# Autodesk Inventor assembly: Ensamblaje carcasa control
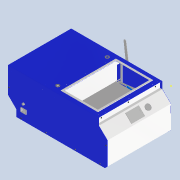
[picture p0: Inventor's stored thumbnail of the model, 180x180]
Saved by Autodesk Inventor 2021 (Build 250183000, 183)
## iProperties
Created: 2021-04-15
Part Number: Ensamblaje carcasa control
Document SubType Name: Assembly
Designer: Admin
Author: Admin
## Documents named in this file (21)
- E:\Documentos\Documentos\Michael_Rodriguez\Universidad_Nacional\Doceaba matricula\PAI\Proyecto PAI\Proyecto_PAI_2021\01 CAD\Ensamblaje carcasa control.iam
- E:\Documentos\Documentos\Michael_Rodriguez\Universidad_Nacional\Doceaba matricula\PAI\Proyecto PAI\Proyecto_PAI_2021\01 CAD\Carcasa_azul.ipt
- E:\Documentos\Documentos\Michael_Rodriguez\Universidad_Nacional\Doceaba matricula\PAI\Proyecto PAI\Proyecto_PAI_2021\01 CAD\Carcaza_blanca_frontal.ipt
- E:\Documentos\Documentos\Michael_Rodriguez\Universidad_Nacional\Doceaba matricula\PAI\Proyecto PAI\Proyecto_PAI_2021\01 CAD\Tapa_blanca_inferior.ipt
- E:\Documentos\Documentos\Michael_Rodriguez\Universidad_Nacional\Doceaba matricula\PAI\Proyecto PAI\Proyecto_PAI_2021\01 CAD\Vacuometro.ipt
- E:\Documentos\Documentos\Michael_Rodriguez\Universidad_Nacional\Doceaba matricula\PAI\Proyecto PAI\Proyecto_PAI_2021\01 CAD\HMI_NV3W_MR20L_V1.iam
- E:\Documentos\Documentos\Michael_Rodriguez\Universidad_Nacional\Doceaba matricula\PAI\Proyecto PAI\Proyecto_PAI_2021\01 CAD\Receptaculo e interruptor.ipt
- E:\Documentos\Documentos\Michael_Rodriguez\Universidad_Nacional\Doceaba matricula\PAI\Proyecto PAI\Proyecto_PAI_2021\01 CAD\Portafusible para fusible de 13A.ipt
- E:\Documentos\Documentos\Michael_Rodriguez\Universidad_Nacional\Doceaba matricula\PAI\Proyecto PAI\Proyecto_PAI_2021\01 CAD\Tapa_interior_1.ipt
- E:\Documentos\Documentos\Michael_Rodriguez\Universidad_Nacional\Doceaba matricula\PAI\Proyecto PAI\Proyecto_PAI_2021\01 CAD\Tapa_interior_2.ipt
- E:\Documentos\Documentos\Michael_Rodriguez\Universidad_Nacional\Doceaba matricula\PAI\Proyecto PAI\Proyecto_PAI_2021\01 CAD\Tapa_blanca_trasera.ipt
- E:\Documentos\Documentos\Michael_Rodriguez\Universidad_Nacional\Doceaba matricula\PAI\Proyecto PAI\Proyecto_PAI_2021\01 CAD\Ensamble eléctrico.iam
- E:\Documentos\Documentos\Michael_Rodriguez\Universidad_Nacional\Doceaba matricula\PAI\Proyecto PAI\Proyecto_PAI_2021\01 CAD\Bomba de Vacio.ipt
- E:\Documentos\Documentos\Michael_Rodriguez\Universidad_Nacional\Doceaba matricula\PAI\Proyecto PAI\Proyecto_PAI_2021\01 CAD\Marco molde.ipt
- E:\Documentos\Documentos\Michael_Rodriguez\Universidad_Nacional\Doceaba matricula\PAI\Proyecto PAI\Proyecto_PAI_2021\01 CAD\CSN 02 1721 - 17,5.ipt
- E:\Documentos\Documentos\Michael_Rodriguez\Universidad_Nacional\Doceaba matricula\PAI\Proyecto PAI\Proyecto_PAI_2021\01 CAD\Ensamblaje_soportme molde_barras.iam
- E:\Documentos\Documentos\Michael_Rodriguez\Universidad_Nacional\Doceaba matricula\PAI\Proyecto PAI\Proyecto_PAI_2021\01 CAD\Mecanismo Modelado.iam
- E:\Documentos\Documentos\Michael_Rodriguez\Universidad_Nacional\Doceaba matricula\PAI\Proyecto PAI\Proyecto_PAI_2021\01 CAD\Bandeja_proteccion_carcasa_control.ipt
- E:\Documentos\Documentos\Michael_Rodriguez\Universidad_Nacional\Doceaba matricula\PAI\Proyecto PAI\Proyecto_PAI_2021\01 CAD\BS 4320 - M5 (Forma A).ipt
- E:\Documentos\Documentos\Michael_Rodriguez\Universidad_Nacional\Doceaba matricula\PAI\Proyecto PAI\Proyecto_PAI_2021\01 CAD\ISO 7380-1 - M5 x 8.ipt
- E:\Documentos\Documentos\Michael_Rodriguez\Universidad_Nacional\Doceaba matricula\PAI\Proyecto PAI\Proyecto_PAI_2021\01 CAD\BS 4183 - M5(1).ipt
## Components (81 placed, 20 different names)
1. Carcasa_azul:1 — Coincidencia:1, Nivelación:1, Coincidencia:2, Coincidencia:3, Nivelación:2, Coincidencia:5, Coincidencia:6, Coincidencia:7, Coincidencia:8, Coincidencia:9, Coincidencia:15, Coincidencia:16, Coincidencia:18, Coincidencia:20, Coincidencia:27, Nivelación:6, Nivelación:7, Coincidencia:28, Coincidencia:29, Coincidencia:30, Coincidencia:31, Coincidencia:32, Coincidencia:33, Coincidencia:34, Nivelación:8, Nivelación:9, Coincidencia:35, De rotación:1, De rotación:2, De rotación:3, De rotación:4, De rotación:5, De rotación:6, De rotación:7, De rotación:8, De rotación:9, De rotación:10, De rotación:11, De rotación:12, De rotación:42, De rotación:43, De rotación:47, De rotación:48
2. Carcaza_blanca_frontal:1 — Coincidencia:1, Nivelación:1, Coincidencia:2, Coincidencia:4, Coincidencia:10, Coincidencia:11, Coincidencia:12, Coincidencia:13, Coincidencia:14, Coincidencia:19, De rotación:24, De rotación:25, De rotación:26, De rotación:56, De rotación:57, De rotación:58
3. Tapa_blanca_inferior:1 — Coincidencia:3, Coincidencia:4, Nivelación:2, Nivelación:4, Coincidencia:21, Mate:25, Flush:5, Mate:26, De rotación:38, De rotación:39, De rotación:40, De rotación:41, De rotación:44, De rotación:45, De rotación:46, De rotación:49, De rotación:50, De rotación:51, De rotación:52, De rotación:53, De rotación:54, De rotación:55
4. Vacuometro:1 — Coincidencia:10, Coincidencia:11
5. HMI_NV3W_MR20L_V1:1 [sub-assembly] — Coincidencia:12, Coincidencia:13, Coincidencia:14
6. Receptaculo e interruptor:1 — Coincidencia:7, Coincidencia:8, Coincidencia:9
7. Portafusible para fusible de 13A:1 — Coincidencia:5, Coincidencia:6
8. Tapa_interior_1:1 — Coincidencia:15, Coincidencia:16, Nivelación:3, Mate:22, Mate:23, Mate:24
9. Tapa_interior_2:1 — Coincidencia:18, Coincidencia:19, Nivelación:3, De rotación:62, De rotación:63, Rígido:1
10. Tapa_blanca_trasera:1 — Coincidencia:20, Nivelación:4, Coincidencia:21, De rotación:32, De rotación:33, De rotación:34
11. Ensamble eléctrico:1 [sub-assembly] — Mate:22, Mate:23, Mate:24
12. Bomba de Vacio:1 — Mate:25, Flush:5, Mate:26
13. Marco molde:1 — Coincidencia:27, Nivelación:6, Nivelación:7
14. CSN 02 1721 17,5:1 — Coincidencia:28, Coincidencia:30, Cilíndrica:1
15. CSN 02 1721 17,5:2 — Coincidencia:29, Coincidencia:31
16. Ensamblaje_soportme molde_barras:1 [sub-assembly] — Cilíndrica:1
17. Mecanismo Modelado:1 [sub-assembly] — Coincidencia:32, Coincidencia:33, Coincidencia:34
18. Bandeja_proteccion_carcasa_control:1 — Nivelación:8, Nivelación:9, Coincidencia:35
19. BS 4320 Forma AB M5 (Forma A):4 — De rotación:1, De rotación:16
20. BS 4320 Forma AB M5 (Forma A):5 — De rotación:2, De rotación:15
21. BS 4320 Forma AB M5 (Forma A):6 — De rotación:3, De rotación:31
22. BS 4320 Forma AB M5 (Forma A):7 — De rotación:4, De rotación:14
23. BS 4320 Forma AB M5 (Forma A):8 — De rotación:5, De rotación:17
24. BS 4320 Forma AB M5 (Forma A):9 — De rotación:6, De rotación:13
25. BS 4320 Forma AB M5 (Forma A):10 — De rotación:9, De rotación:21
26. BS 4320 Forma AB M5 (Forma A):11 — De rotación:7, De rotación:23
27. BS 4320 Forma AB M5 (Forma A):12 — De rotación:11, De rotación:19
28. BS 4320 Forma AB M5 (Forma A):13 — De rotación:8, De rotación:22
29. BS 4320 Forma AB M5 (Forma A):14 — De rotación:10, De rotación:20
30. BS 4320 Forma AB M5 (Forma A):15 — De rotación:12, De rotación:30
31. ISO 7380-1 M5 x 8:1 — De rotación:15
32. ISO 7380-1 M5 x 8:3 — De rotación:17
33. ISO 7380-1 M5 x 8:4 — De rotación:16
34. ISO 7380-1 M5 x 8:5 — De rotación:14
35. ISO 7380-1 M5 x 8:6 — De rotación:13
36. ISO 7380-1 M5 x 8:7 — De rotación:20
37. ISO 7380-1 M5 x 8:8 — De rotación:21
38. ISO 7380-1 M5 x 8:10 — De rotación:23
39. ISO 7380-1 M5 x 8:11 — De rotación:19
40. ISO 7380-1 M5 x 8:12 — De rotación:22
41. ISO 7380-1 M5 x 8:13 — De rotación:27
42. ISO 7380-1 M5 x 8:14 — De rotación:29
43. ISO 7380-1 M5 x 8:15 — De rotación:28
44. BS 4320 Forma AB M5 (Forma A):16 — De rotación:26, De rotación:27
45. BS 4320 Forma AB M5 (Forma A):17 — De rotación:25, De rotación:28
46. BS 4320 Forma AB M5 (Forma A):18 — De rotación:24, De rotación:29
47. ISO 7380-1 M5 x 8:16 — De rotación:30
48. ISO 7380-1 M5 x 8:17 — De rotación:31
49. ISO 7380-1 M5 x 8:18 — De rotación:35
50. ISO 7380-1 M5 x 8:19 — De rotación:36
51. ISO 7380-1 M5 x 8:20 — De rotación:37
52. BS 4320 Forma AB M5 (Forma A):19 — De rotación:32, De rotación:35
53. BS 4320 Forma AB M5 (Forma A):20 — De rotación:33, De rotación:36
54. BS 4320 Forma AB M5 (Forma A):21 — De rotación:34, De rotación:37
55. BS 4183 - Métrico M5:1 — De rotación:38
56. BS 4183 - Métrico M5:2 — De rotación:39
57. BS 4183 - Métrico M5:3 — De rotación:42
58. BS 4183 - Métrico M5:4 — De rotación:40
59. BS 4183 - Métrico M5:5 — De rotación:43
60. BS 4183 - Métrico M5:6 — De rotación:41
61. BS 4183 - Métrico M5:7 — De rotación:45
62. BS 4183 - Métrico M5:8 — De rotación:44
63. BS 4183 - Métrico M5:9 — De rotación:47
64. BS 4183 - Métrico M5:10 — De rotación:46
65. BS 4183 - Métrico M5:11 — De rotación:48
66. BS 4183 - Métrico M5:12 — De rotación:49
67. BS 4183 - Métrico M5:13 — De rotación:50
68. BS 4183 - Métrico M5:14 — De rotación:52
69. BS 4183 - Métrico M5:15 — De rotación:51
70. BS 4183 - Métrico M5:16 — De rotación:54
71. BS 4183 - Métrico M5:17 — De rotación:53
72. BS 4183 - Métrico M5:18 — De rotación:55
73. ISO 7380-1 M5 x 8:21 — De rotación:59
74. ISO 7380-1 M5 x 8:22 — De rotación:60
75. ISO 7380-1 M5 x 8:23 — De rotación:61
76. BS 4320 Forma AB M5 (Forma A):22 — De rotación:57, De rotación:60
77. BS 4320 Forma AB M5 (Forma A):23 — De rotación:58, De rotación:61
78. BS 4320 Forma AB M5 (Forma A):24 — De rotación:56, De rotación:59
79. BS 4183 - Métrico M5:19 — De rotación:62
80. BS 4183 - Métrico M5:20 — De rotación:63
81. BS 4183 - Métrico M5:21 — Rígido:1
## Relationships (107: RevoluteJoint 62, Mate 34, Flush 9, CylindricalJoint 1, WeldJoint 1)
- Coincidencia:1 [Mate]: Carcasa_azul:1 ↔ Carcaza_blanca_frontal:1
- Nivelación:1 [Flush]: Carcasa_azul:1 ↔ Carcaza_blanca_frontal:1
- Coincidencia:2 [Mate]: Carcasa_azul:1 ↔ Carcaza_blanca_frontal:1
- Coincidencia:3 [Mate]: Carcasa_azul:1 ↔ Tapa_blanca_inferior:1
- Coincidencia:4 [Mate]: Carcaza_blanca_frontal:1 ↔ Tapa_blanca_inferior:1
- Nivelación:2 [Flush]: Carcasa_azul:1 ↔ Tapa_blanca_inferior:1
- Coincidencia:5 [Mate]: Carcasa_azul:1 ↔ Portafusible para fusible de 13A:1
- Coincidencia:6 [Mate]: Carcasa_azul:1 ↔ Portafusible para fusible de 13A:1
- Coincidencia:7 [Mate]: Carcasa_azul:1 ↔ Receptaculo e interruptor:1
- Coincidencia:8 [Mate]: Carcasa_azul:1 ↔ Receptaculo e interruptor:1
- Coincidencia:9 [Mate]: Carcasa_azul:1 ↔ Receptaculo e interruptor:1
- Coincidencia:10 [Mate]: Carcaza_blanca_frontal:1 ↔ Vacuometro:1
- Coincidencia:11 [Mate]: Carcaza_blanca_frontal:1 ↔ Vacuometro:1
- Coincidencia:12 [Mate]: Carcaza_blanca_frontal:1 ↔ HMI_NV3W_MR20L_V1:1
- Coincidencia:13 [Mate]: Carcaza_blanca_frontal:1 ↔ HMI_NV3W_MR20L_V1:1
- Coincidencia:14 [Mate]: Carcaza_blanca_frontal:1 ↔ HMI_NV3W_MR20L_V1:1
- Coincidencia:15 [Mate]: Carcasa_azul:1 ↔ Tapa_interior_1:1
- Coincidencia:16 [Mate] (20 mm): Carcasa_azul:1 ↔ Tapa_interior_1:1
- Coincidencia:18 [Mate]: Carcasa_azul:1 ↔ Tapa_interior_2:1
- Coincidencia:19 [Mate]: Carcaza_blanca_frontal:1 ↔ Tapa_interior_2:1
- Nivelación:3 [Flush]: Tapa_interior_1:1 ↔ Tapa_interior_2:1
- Coincidencia:20 [Mate]: Carcasa_azul:1 ↔ Tapa_blanca_trasera:1
- Nivelación:4 [Flush]: Tapa_blanca_inferior:1 ↔ Tapa_blanca_trasera:1
- Coincidencia:21 [Mate]: Tapa_blanca_inferior:1 ↔ Tapa_blanca_trasera:1
- Mate:22: Tapa_interior_1:1 ↔ Ensamble eléctrico:1
- Mate:23: Tapa_interior_1:1 ↔ Ensamble eléctrico:1
- Mate:24: Tapa_interior_1:1 ↔ Ensamble eléctrico:1
- Mate:25: Tapa_blanca_inferior:1 ↔ Bomba de Vacio:1
- Flush:5 (70 mm): Tapa_blanca_inferior:1 ↔ Bomba de Vacio:1
- Mate:26 (130 mm): Tapa_blanca_inferior:1 ↔ Bomba de Vacio:1
- Coincidencia:27 [Mate]: Carcasa_azul:1 ↔ Marco molde:1
- Nivelación:6 [Flush]: Carcasa_azul:1 ↔ Marco molde:1
- Nivelación:7 [Flush]: Carcasa_azul:1 ↔ Marco molde:1
- Coincidencia:28 [Mate]: Carcasa_azul:1 ↔ CSN 02 1721 17,5:1
- Coincidencia:29 [Mate]: Carcasa_azul:1 ↔ CSN 02 1721 17,5:2
- Coincidencia:30 [Mate]: Carcasa_azul:1 ↔ CSN 02 1721 17,5:1
- Coincidencia:31 [Mate]: Carcasa_azul:1 ↔ CSN 02 1721 17,5:2
- Cilíndrica:1 [CylindricalJoint]: CSN 02 1721 17,5:1 ↔ Ensamblaje_soportme molde_barras:1
- Coincidencia:32 [Mate]: Carcasa_azul:1 ↔ Mecanismo Modelado:1
- Coincidencia:33 [Mate]: Carcasa_azul:1 ↔ Mecanismo Modelado:1
- Coincidencia:34 [Mate]: Carcasa_azul:1 ↔ Mecanismo Modelado:1
- Nivelación:8 [Flush] (5 mm): Carcasa_azul:1 ↔ Bandeja_proteccion_carcasa_control:1
- Nivelación:9 [Flush]: Carcasa_azul:1 ↔ Bandeja_proteccion_carcasa_control:1
- Coincidencia:35 [Mate]: Carcasa_azul:1 ↔ Bandeja_proteccion_carcasa_control:1
- De rotación:1 [RevoluteJoint]: Carcasa_azul:1 ↔ BS 4320 Forma AB M5 (Forma A):4
- De rotación:2 [RevoluteJoint]: Carcasa_azul:1 ↔ BS 4320 Forma AB M5 (Forma A):5
- De rotación:3 [RevoluteJoint]: Carcasa_azul:1 ↔ BS 4320 Forma AB M5 (Forma A):6
- De rotación:4 [RevoluteJoint]: Carcasa_azul:1 ↔ BS 4320 Forma AB M5 (Forma A):7
- De rotación:5 [RevoluteJoint]: Carcasa_azul:1 ↔ BS 4320 Forma AB M5 (Forma A):8
- De rotación:6 [RevoluteJoint]: Carcasa_azul:1 ↔ BS 4320 Forma AB M5 (Forma A):9
- De rotación:7 [RevoluteJoint]: Carcasa_azul:1 ↔ BS 4320 Forma AB M5 (Forma A):11
- De rotación:8 [RevoluteJoint]: Carcasa_azul:1 ↔ BS 4320 Forma AB M5 (Forma A):13
- De rotación:9 [RevoluteJoint]: Carcasa_azul:1 ↔ BS 4320 Forma AB M5 (Forma A):10
- De rotación:10 [RevoluteJoint]: Carcasa_azul:1 ↔ BS 4320 Forma AB M5 (Forma A):14
- De rotación:11 [RevoluteJoint]: Carcasa_azul:1 ↔ BS 4320 Forma AB M5 (Forma A):12
- De rotación:12 [RevoluteJoint]: Carcasa_azul:1 ↔ BS 4320 Forma AB M5 (Forma A):15
- De rotación:13 [RevoluteJoint]: BS 4320 Forma AB M5 (Forma A):9 ↔ ISO 7380-1 M5 x 8:6
- De rotación:14 [RevoluteJoint]: BS 4320 Forma AB M5 (Forma A):7 ↔ ISO 7380-1 M5 x 8:5
- De rotación:15 [RevoluteJoint]: BS 4320 Forma AB M5 (Forma A):5 ↔ ISO 7380-1 M5 x 8:1
- De rotación:16 [RevoluteJoint]: BS 4320 Forma AB M5 (Forma A):4 ↔ ISO 7380-1 M5 x 8:4
- De rotación:17 [RevoluteJoint]: BS 4320 Forma AB M5 (Forma A):8 ↔ ISO 7380-1 M5 x 8:3
- De rotación:19 [RevoluteJoint]: BS 4320 Forma AB M5 (Forma A):12 ↔ ISO 7380-1 M5 x 8:11
- De rotación:20 [RevoluteJoint]: BS 4320 Forma AB M5 (Forma A):14 ↔ ISO 7380-1 M5 x 8:7
- De rotación:21 [RevoluteJoint]: BS 4320 Forma AB M5 (Forma A):10 ↔ ISO 7380-1 M5 x 8:8
- De rotación:22 [RevoluteJoint]: BS 4320 Forma AB M5 (Forma A):13 ↔ ISO 7380-1 M5 x 8:12
- De rotación:23 [RevoluteJoint]: BS 4320 Forma AB M5 (Forma A):11 ↔ ISO 7380-1 M5 x 8:10
- De rotación:24 [RevoluteJoint]: Carcaza_blanca_frontal:1 ↔ BS 4320 Forma AB M5 (Forma A):18
- De rotación:25 [RevoluteJoint]: Carcaza_blanca_frontal:1 ↔ BS 4320 Forma AB M5 (Forma A):17
- De rotación:26 [RevoluteJoint]: Carcaza_blanca_frontal:1 ↔ BS 4320 Forma AB M5 (Forma A):16
- De rotación:27 [RevoluteJoint]: ISO 7380-1 M5 x 8:13 ↔ BS 4320 Forma AB M5 (Forma A):16
- De rotación:28 [RevoluteJoint]: ISO 7380-1 M5 x 8:15 ↔ BS 4320 Forma AB M5 (Forma A):17
- De rotación:29 [RevoluteJoint]: ISO 7380-1 M5 x 8:14 ↔ BS 4320 Forma AB M5 (Forma A):18
- De rotación:30 [RevoluteJoint]: BS 4320 Forma AB M5 (Forma A):15 ↔ ISO 7380-1 M5 x 8:16
- De rotación:31 [RevoluteJoint]: BS 4320 Forma AB M5 (Forma A):6 ↔ ISO 7380-1 M5 x 8:17
- De rotación:32 [RevoluteJoint]: Tapa_blanca_trasera:1 ↔ BS 4320 Forma AB M5 (Forma A):19
- De rotación:33 [RevoluteJoint]: Tapa_blanca_trasera:1 ↔ BS 4320 Forma AB M5 (Forma A):20
- De rotación:34 [RevoluteJoint]: Tapa_blanca_trasera:1 ↔ BS 4320 Forma AB M5 (Forma A):21
- De rotación:35 [RevoluteJoint]: ISO 7380-1 M5 x 8:18 ↔ BS 4320 Forma AB M5 (Forma A):19
- De rotación:36 [RevoluteJoint]: ISO 7380-1 M5 x 8:19 ↔ BS 4320 Forma AB M5 (Forma A):20
- De rotación:37 [RevoluteJoint]: ISO 7380-1 M5 x 8:20 ↔ BS 4320 Forma AB M5 (Forma A):21
- De rotación:38 [RevoluteJoint]: Tapa_blanca_inferior:1 ↔ BS 4183 - Métrico M5:1
- De rotación:39 [RevoluteJoint]: Tapa_blanca_inferior:1 ↔ BS 4183 - Métrico M5:2
- De rotación:40 [RevoluteJoint]: Tapa_blanca_inferior:1 ↔ BS 4183 - Métrico M5:4
- De rotación:41 [RevoluteJoint]: Tapa_blanca_inferior:1 ↔ BS 4183 - Métrico M5:6
- De rotación:42 [RevoluteJoint]: Carcasa_azul:1 ↔ BS 4183 - Métrico M5:3
- De rotación:43 [RevoluteJoint]: Carcasa_azul:1 ↔ BS 4183 - Métrico M5:5
- De rotación:44 [RevoluteJoint]: Tapa_blanca_inferior:1 ↔ BS 4183 - Métrico M5:8
- De rotación:45 [RevoluteJoint]: Tapa_blanca_inferior:1 ↔ BS 4183 - Métrico M5:7
- De rotación:46 [RevoluteJoint]: Tapa_blanca_inferior:1 ↔ BS 4183 - Métrico M5:10
- De rotación:47 [RevoluteJoint]: Carcasa_azul:1 ↔ BS 4183 - Métrico M5:9
- De rotación:48 [RevoluteJoint]: Carcasa_azul:1 ↔ BS 4183 - Métrico M5:11
- De rotación:49 [RevoluteJoint]: Tapa_blanca_inferior:1 ↔ BS 4183 - Métrico M5:12
- De rotación:50 [RevoluteJoint]: Tapa_blanca_inferior:1 ↔ BS 4183 - Métrico M5:13
- De rotación:51 [RevoluteJoint]: Tapa_blanca_inferior:1 ↔ BS 4183 - Métrico M5:15
- De rotación:52 [RevoluteJoint]: Tapa_blanca_inferior:1 ↔ BS 4183 - Métrico M5:14
- De rotación:53 [RevoluteJoint]: Tapa_blanca_inferior:1 ↔ BS 4183 - Métrico M5:17
- De rotación:54 [RevoluteJoint]: Tapa_blanca_inferior:1 ↔ BS 4183 - Métrico M5:16
- De rotación:55 [RevoluteJoint]: Tapa_blanca_inferior:1 ↔ BS 4183 - Métrico M5:18
- De rotación:56 [RevoluteJoint]: Carcaza_blanca_frontal:1 ↔ BS 4320 Forma AB M5 (Forma A):24
- De rotación:57 [RevoluteJoint]: Carcaza_blanca_frontal:1 ↔ BS 4320 Forma AB M5 (Forma A):22
- De rotación:58 [RevoluteJoint]: Carcaza_blanca_frontal:1 ↔ BS 4320 Forma AB M5 (Forma A):23
- De rotación:59 [RevoluteJoint]: ISO 7380-1 M5 x 8:21 ↔ BS 4320 Forma AB M5 (Forma A):24
- De rotación:60 [RevoluteJoint]: ISO 7380-1 M5 x 8:22 ↔ BS 4320 Forma AB M5 (Forma A):22
- De rotación:61 [RevoluteJoint]: ISO 7380-1 M5 x 8:23 ↔ BS 4320 Forma AB M5 (Forma A):23
- De rotación:62 [RevoluteJoint]: Tapa_interior_2:1 ↔ BS 4183 - Métrico M5:19
- De rotación:63 [RevoluteJoint]: Tapa_interior_2:1 ↔ BS 4183 - Métrico M5:20
- Rígido:1 [WeldJoint]: Tapa_interior_2:1 ↔ BS 4183 - Métrico M5:21
